# Autodesk Inventor assembly: 193995 DSNU-63-500-P-A---(500PA---00--0-------0)
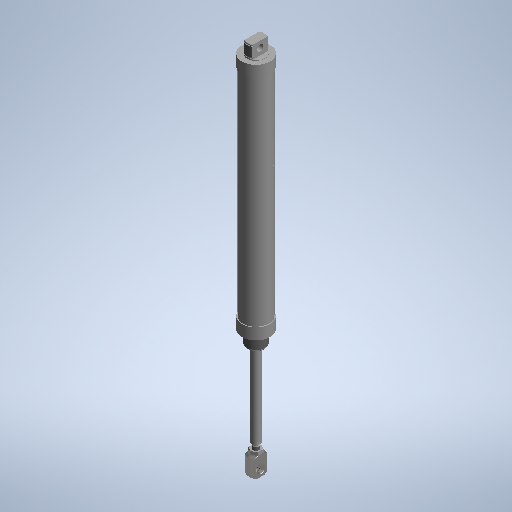
[picture p0: Inventor's stored thumbnail of the model, 512x512]
Saved by Autodesk Inventor 2025.2 (Build 292293000, 293)
## iProperties
Category: PARTsolutions
Company: FESTO
Part Number: 193995 DSNU-63-500-P-A---(500PA---00--0-------0)
Catalog Web Link: www.cadenas.de
Description: DSNU (m)-Round cylinder, Modular system
Vendor: FESTO
Document SubType Name: Assembly
Designer: partserver
Manufacturer: FESTO
Mass: 719.326 g
Surface Area: 3103.34 cm^2
Volume: 719.326 cm^3
Density: 1 g/cm^3
PSOL_IDENT_0: {ATYP=ASSISTANT},{DATA=script=$CADENAS_DATA/23d-libs/festo/webfesto.vbb/&M_FAMILY=DSNU&M_GROUP=01&M_
PSOL_IDENT_1: PARTNO=193995&IDCODE1=DSNU-63-500-P-A&IDCODE2=&C_DSNU_DM=63&C_DSNU_HEAD=DSNU&HUB=500&M_AA=A&M_DAA=P&
PSOL_IDENT_2: S_SMS=N&VCSD_UPDATE_YYIDENT11=DSNU-63-500-P-A&customer_number_cns=&MATES=1&LOD=HI&LOCKERP=1}
NB: 193995 DSNU-63-500-P-A---(500PA---00--0-------0)
NN: DSNU (m)
NT: Round cylinder, Modular system
NBSYN: $TNR. $IDCODE1.---($HUB.$DA.$PE.$ZD.$VS.$KA.$K2A.$K6.$K3.$K5.$K8.$KP.$R3.$R8.$TB.$KS.$LS.$ATEX.$HUBST.)
LINA: 193995 DSNU-63-500-P-A
CATALOG: Festo
OFFICIAL_STANDARD_NUMBERS: ISO 6432
TNR: 193995
TYP: DSNU-63
KDM: 63
HUB: 500
HUBST: 0
DA: P
PE: A
ZD: -
VS: -
KA: -
K2A: 0
K6: 0
K3: -
K5: -
K8: 0
KP: -
R3: -
R8: -
TB: -
KS: -
LS: -
ATEX: -
A1: 70
A2: 500
A3: 10
A4: 87.5
AB: 44
AM: 32
B: 45
BB: 4
BE: M45x1,5
BS: 11
B1: 72
B2: 17
B3: 44
B4: 15
B5: 36
B6: 18
B7: 4
CD: 16
D: 70
D1: 45
D2: 20
D3: 65.4
D4: 16
D5: 66
D6: 60
D7: 45
EE: G3/8
EW: 21
F: 52
FF: M8
F1: 36
H: 72
H1: 8
KK: M16x1.5
K1: M10
K2: 3.5
KV: 0
KW: 10
KV2: 24
KW2: 8
L: 16
LH: 15
LK: 28
L1: 672.2
L2: 594.2
L3: 13
L4: 33
L5: 30
L6: 77
L7: 44
L8: 28
L9: 32
L10: 117.2
L11: 132.2
L12: 94.2
L13: 184.2
ST: 11
SW: 17
T: 16
WH: 45
X: 4.7
XC: 656.2
SUPPLIER: FESTO
ARTICLENO: 193995 DSNU-63-500-P-A---(500PA---00--0-------0)
BOMINFO: 193995 DSNU-63-500-P-A
CREATOR: CADENAS GmbH
Title: 193995 DSNU-63-500-P-A
Author: Cadenas PARTsolutions
Comments: Round cylinder, Modular system
## Documents named in this file (5)
- C:\Users\Victor\Documents\LineFollowerRobot\Anomaly_Detection\Mechanical_Project\Inventor_project\193995 DSNU-63-500-P-A---(500PA---00--0-------0).iam
- C:\Users\Victor\Documents\LineFollowerRobot\Anomaly_Detection\Mechanical_Project\Inventor_project\193995 DSNU-63-500-P---(A----0-ZR).ipt
- C:\Users\Victor\Documents\LineFollowerRobot\Anomaly_Detection\Mechanical_Project\Inventor_project\193995 DSNU-63-500-P---(A---00--0-KS).ipt
- C:\Users\Victor\Documents\LineFollowerRobot\Anomaly_Detection\Mechanical_Project\Inventor_project\DIN-439-B - M16x1_5(F).ipt
- C:\Users\Victor\Documents\LineFollowerRobot\Anomaly_Detection\Mechanical_Project\Inventor_project\IMS-01-002.ipt
## Components (4 placed, 4 different names)
1. 193995 DSNU-63-500-P---(A----0-ZR):1 — ZR_Z@1 <-> KS_Z@3, ZR_YZ@1 <-> KS_YZ@3, Angle:3
2. 193995 DSNU-63-500-P---(A---00--0-KS):1 — ZR_Z@1 <-> KS_Z@3, ZR_YZ@1 <-> KS_YZ@3, NUT1_XY@3 <-> 2CYL_XY@4, NUT1_Z@3 <-> 2CYL_Z@4, NUT1_YZ@3 <-> 2CYL_YZ@4, Mate:5
3. DIN-439-B - M16x1_5(F):1 — NUT1_XY@3 <-> 2CYL_XY@4, NUT1_Z@3 <-> 2CYL_Z@4, NUT1_YZ@3 <-> 2CYL_YZ@4, Mate:6
4. IMS-01-002:1 — Mate:5, Mate:6, Angle:3
## Relationships (8: Mate 5, Angle 3)
- ZR_Z@1 <-> KS_Z@3 [Mate]: 193995 DSNU-63-500-P---(A----0-ZR):1 ↔ 193995 DSNU-63-500-P---(A---00--0-KS):1
- ZR_YZ@1 <-> KS_YZ@3 [Angle] (0 deg): 193995 DSNU-63-500-P---(A----0-ZR):1 ↔ 193995 DSNU-63-500-P---(A---00--0-KS):1
- NUT1_XY@3 <-> 2CYL_XY@4 [Mate] (-4 mm): 193995 DSNU-63-500-P---(A---00--0-KS):1 ↔ DIN-439-B - M16x1_5(F):1
- NUT1_Z@3 <-> 2CYL_Z@4 [Mate]: 193995 DSNU-63-500-P---(A---00--0-KS):1 ↔ DIN-439-B - M16x1_5(F):1
- NUT1_YZ@3 <-> 2CYL_YZ@4 [Angle] (0 deg): 193995 DSNU-63-500-P---(A---00--0-KS):1 ↔ DIN-439-B - M16x1_5(F):1
- Mate:5: 193995 DSNU-63-500-P---(A---00--0-KS):1 ↔ IMS-01-002:1
- Mate:6: DIN-439-B - M16x1_5(F):1 ↔ IMS-01-002:1
- Angle:3 (0 deg): 193995 DSNU-63-500-P---(A----0-ZR):1 ↔ IMS-01-002:1
